# Autodesk Inventor assembly: right
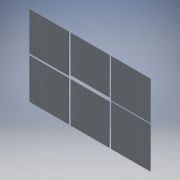
[picture p0: Inventor's stored thumbnail of the model, 180x180]
Saved by Autodesk Inventor 2019 (Build 230136000, 136)
## iProperties
Created: 2018-07-10
Part Number: right
Document SubType Name: Assembly
Designer: User
Author: User
## Documents named in this file (7)
- C:\Users\User\Desktop\Room Model\right.iam
- C:\Users\User\Desktop\Room Model\right_0_0.ipt
- C:\Users\User\Desktop\Room Model\right_0_1.ipt
- C:\Users\User\Desktop\Room Model\right_0_2.ipt
- C:\Users\User\Desktop\Room Model\right_1_0.ipt
- C:\Users\User\Desktop\Room Model\right_1_1.ipt
- C:\Users\User\Desktop\Room Model\right_1_2.ipt
## Components (6 placed, 6 different names)
1. right_0_0:1 — Rigid:1
2. right_0_1:1 — Rigid:1, Rigid:2, Rigid:4
3. right_0_2:1 — Rigid:2
4. right_1_0:1 — Rigid:3
5. right_1_1:1 — Rigid:3, Rigid:4, Rigid:5
6. right_1_2:1 — Rigid:5
## Relationships (5: WeldJoint 5)
- Rigid:1 [WeldJoint] (57.15 mm): right_0_0:1 ↔ right_0_1:1
- Rigid:2 [WeldJoint] (53.975 mm): right_0_1:1 ↔ right_0_2:1
- Rigid:3 [WeldJoint] (57.15 mm): right_1_0:1 ↔ right_1_1:1
- Rigid:4 [WeldJoint] (101.6 mm): right_0_1:1 ↔ right_1_1:1
- Rigid:5 [WeldJoint] (53.975 mm): right_1_1:1 ↔ right_1_2:1
